# Autodesk Inventor assembly: Injector assembly
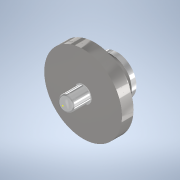
[picture p0: Inventor's stored thumbnail of the model, 180x180]
Saved by Autodesk Inventor 2021 (Build 250183000, 183)
## iProperties
Created: 2022-08-16
Part Number: Injector assembly
Document SubType Name: Assembly
Designer: pc
Mass: 4985.89 g
Surface Area: 1591.37 cm^2
Volume: 747.517 cm^3
Density: 6.66994 g/cm^3
Author: pc
## Documents named in this file (6)
- C:\Users\pc\Documents\injector\Injector assembly.iam
- C:\Users\pc\Documents\injector\Part1.ipt
- C:\Users\pc\Documents\injector\Orifice Plate.ipt
- C:\Users\pc\Documents\injector\faceplate.ipt
- C:\Users\pc\Documents\injector\pintle body.ipt
- C:\Users\pc\Documents\injector\Pintle tip.ipt
## Components (5 placed, 5 different names)
1. Orifice Plate:1 — Mate:1, Rotational:1
2. Part1:1 — Mate:1, Rotational:1, Mate:2, Rotational:2, Mate:3, Rigid:1, Mate:4
3. faceplate:2 — Mate:2, Rotational:2
4. pintle body:1 — Mate:3, Rigid:1, Rotational:3
5. Pintle tip:1 — Mate:4, Rotational:3
## Relationships (8: Mate 4, RevoluteJoint 3, WeldJoint 1)
- Mate:1: Orifice Plate:1 ↔ Part1:1
- Rotational:1 [RevoluteJoint]: Orifice Plate:1 ↔ Part1:1
- Mate:2: Part1:1 ↔ faceplate:2
- Rotational:2 [RevoluteJoint]: Part1:1 ↔ faceplate:2
- Mate:3: Part1:1 ↔ pintle body:1
- Rigid:1 [WeldJoint]: Part1:1 ↔ pintle body:1
- Mate:4: Part1:1 ↔ Pintle tip:1
- Rotational:3 [RevoluteJoint]: pintle body:1 ↔ Pintle tip:1
